# Autodesk Inventor assembly: assembly_full
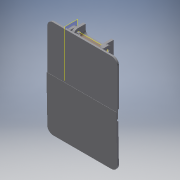
[picture p0: Inventor's stored thumbnail of the model, 180x180]
Saved by Autodesk Inventor 2017 (Build 210142000, 142)
## iProperties
Created: 2017-06-21
Part Number: assembly_full
Document SubType Name: Assembly
Designer: erwin
Author: erwin
## Documents named in this file (7)
- D:\Erwin\OneDrive\Projects\RepRap\Office Coffee Disposal Monitor\assembly_full.iam
- D:\Erwin\OneDrive\Projects\RepRap\Office Coffee Disposal Monitor\top_right.ipt
- D:\Erwin\OneDrive\Projects\RepRap\Office Coffee Disposal Monitor\base.ipt
- D:\Erwin\OneDrive\Projects\RepRap\Office Coffee Disposal Monitor\fastener.ipt
- D:\Erwin\OneDrive\Projects\RepRap\Office Coffee Disposal Monitor\tensioner.ipt
- D:\Erwin\OneDrive\Dualog\Garage\NoGoFish\proto1\Case_Improved\aaa.ipt
- D:\Erwin\OneDrive\Dualog\Garage\NoGoFish\proto1\Case_Improved\cover_new.ipt
## Components (7 placed, 6 different names)
1. top_right:1 — Mate:1, Rotational:1, Flush:3, Flush:7, Flush:8
2. base:1 — Mate:1, Rotational:1, Flush:3, Rotational:2, Flush:9, Flush:10, Flush:11, Flush:12
3. top_right:2 — Rotational:2
4. fastener:1 — Flush:7, Flush:8
5. tensioner:1 — Flush:9
6. aaa:1 — Flush:10
7. cover_new:1 — Flush:11, Flush:12
## Relationships (10: Flush 7, RevoluteJoint 2, Mate 1)
- Mate:1: top_right:1 ↔ base:1
- Rotational:1 [RevoluteJoint]: top_right:1 ↔ base:1
- Flush:3: top_right:1 ↔ base:1
- Rotational:2 [RevoluteJoint]: base:1 ↔ top_right:2
- Flush:7: top_right:1 ↔ fastener:1
- Flush:8: top_right:1 ↔ fastener:1
- Flush:9: base:1 ↔ tensioner:1
- Flush:10: base:1 ↔ aaa:1
- Flush:11: base:1 ↔ cover_new:1
- Flush:12: base:1 ↔ cover_new:1
